# Autodesk Inventor assembly: CamRight
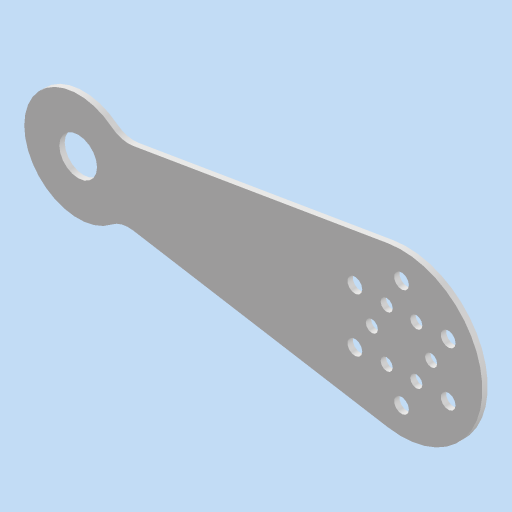
[picture p0: Inventor's stored thumbnail of the model, 512x512]
Saved by Autodesk Inventor 2023 (Build 270158000, 158)
## iProperties
Created: 2026-05-26
Part Number: CamRight
Document SubType Name: Assembly
Designer: Nathann
Author: Nathann
Revision Number: ANY
## Documents named in this file (2)
- C:\Users\Nathann\OneDrive\ClawdDrive\Objet3D\RunningRobot\PartURDF\CamRight.iam
- C:\Users\Nathann\OneDrive\ClawdDrive\Objet3D\RunningRobot\testfour_bar_bend_Défaut.ipt
## Components (1 placed, 1 different names)
1. four_bar_bend_Défaut_342 — Mate:1, Mate:2, Flush:1
## Relationships (3: Mate 2, Flush 1)
- Mate:1: four_bar_bend_Défaut_342
- Mate:2: four_bar_bend_Défaut_342
- Flush:1: four_bar_bend_Défaut_342
